# Autodesk Inventor assembly: LEGO Stair Assembly
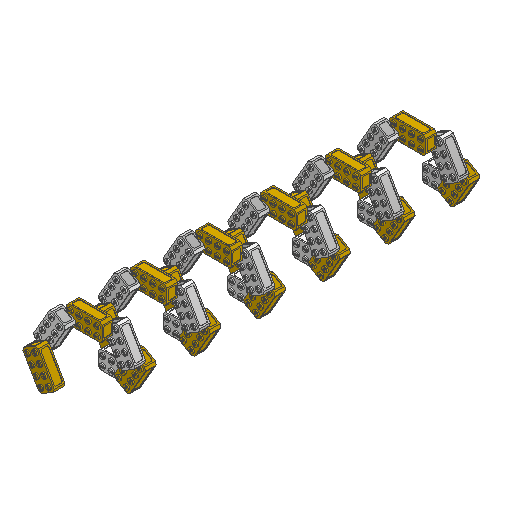
[picture p0: Inventor's stored thumbnail of the model, 512x512]
Saved by Autodesk Inventor 2026.2 (Build 302298000, 298)
## iProperties
Created: 2026-01-27
Part Number: LEGO Stair Assembly
Document SubType Name: Assembly
Designer: andyeske
Author: andyeske
## Documents named in this file (2)
- C:\Users\andyeske\Inventor\LEGO Stair Assembly.iam
- C:\Users\andyeske\Inventor\CAD 2x4 Brick.ipt
## Components (36 placed, 1 different names)
1. CAD 2x4 Brick:6
2. CAD 2x4 Brick:5
3. CAD 2x4 Brick:4 — Cylindrical:5, Mate:5, Angle:5
4. CAD 2x4 Brick:3 — Cylindrical:2, Mate:2, Angle:2, Cylindrical:5, Mate:5, Angle:5
5. CAD 2x4 Brick:2 — Cylindrical:1, Mate:1, Angle:1, Cylindrical:2, Mate:2, Angle:2
6. CAD 2x4 Brick:1 — Cylindrical:1, Mate:1, Angle:1
7. CAD 2x4 Brick:7
8. CAD 2x4 Brick:8
9. CAD 2x4 Brick:9
10. CAD 2x4 Brick:10
11. CAD 2x4 Brick:11
12. CAD 2x4 Brick:12
13. CAD 2x4 Brick:13
14. CAD 2x4 Brick:14
15. CAD 2x4 Brick:15
16. CAD 2x4 Brick:16
17. CAD 2x4 Brick:17
18. CAD 2x4 Brick:18
19. CAD 2x4 Brick:19
20. CAD 2x4 Brick:20
21. CAD 2x4 Brick:21
22. CAD 2x4 Brick:22
23. CAD 2x4 Brick:23
24. CAD 2x4 Brick:24
25. CAD 2x4 Brick:25
26. CAD 2x4 Brick:26
27. CAD 2x4 Brick:27
28. CAD 2x4 Brick:28
29. CAD 2x4 Brick:29
30. CAD 2x4 Brick:30
31. CAD 2x4 Brick:31
32. CAD 2x4 Brick:32
33. CAD 2x4 Brick:33
34. CAD 2x4 Brick:34
35. CAD 2x4 Brick:35
36. CAD 2x4 Brick:36
## Component patterns: (6 elements, first: CAD 2x4 Brick:6 + CAD 2x4 Brick:5 + CAD 2x4 Brick:4 + CAD 2x4 Brick:3 + CAD 2x4 Brick:2 + CAD 2x4 Brick:1)
## Relationships (15: CylindricalJoint 5, Mate 5, Angle 5)
- Cylindrical:1: CAD 2x4 Brick:2 ↔ CAD 2x4 Brick:1
- Mate:1: CAD 2x4 Brick:2 ↔ CAD 2x4 Brick:1
- Angle:1 (300 deg): CAD 2x4 Brick:2 ↔ CAD 2x4 Brick:1
- Cylindrical:2: CAD 2x4 Brick:3 ↔ CAD 2x4 Brick:2
- Mate:2: CAD 2x4 Brick:3 ↔ CAD 2x4 Brick:2
- Angle:2 (300 deg): CAD 2x4 Brick:3 ↔ CAD 2x4 Brick:2
- [CylindricalJoint]: CAD 2x4 Brick:5 ↔ CAD 2x4 Brick:4
- [Mate]: CAD 2x4 Brick:5 ↔ CAD 2x4 Brick:4
- [Angle] (300 deg): CAD 2x4 Brick:5 ↔ CAD 2x4 Brick:4
- [CylindricalJoint]: CAD 2x4 Brick:6 ↔ CAD 2x4 Brick:5
- [Mate]: CAD 2x4 Brick:6 ↔ CAD 2x4 Brick:5
- [Angle] (300 deg): CAD 2x4 Brick:6 ↔ CAD 2x4 Brick:5
- Cylindrical:5: CAD 2x4 Brick:4 ↔ CAD 2x4 Brick:3
- Mate:5: CAD 2x4 Brick:4 ↔ CAD 2x4 Brick:3
- Angle:5 (300 deg): CAD 2x4 Brick:4 ↔ CAD 2x4 Brick:3
## Named parameters: d40_d35 = 300 deg, d41_d36 = 60 deg, d42_d37 = 8.4 mm, d43_d38 = 0 mm, d44_d39 = 300 deg, d45_d32 = -120 deg, d46_d33 = 9.6 mm, d47_d34 = 0 mm, Finish3_Area = 650.804, Finish4_Area = 38.2826, Finish5_Area = 76.5652, Finish6_Area = 76.5652
note: some values were not read from the file. Shown as the stored number, unit unknown: "Finish3_Area", "Finish4_Area", "Finish5_Area", "Finish6_Area".
